# Autodesk Inventor assembly: Servo-Arm-20mm-Ball-Joint
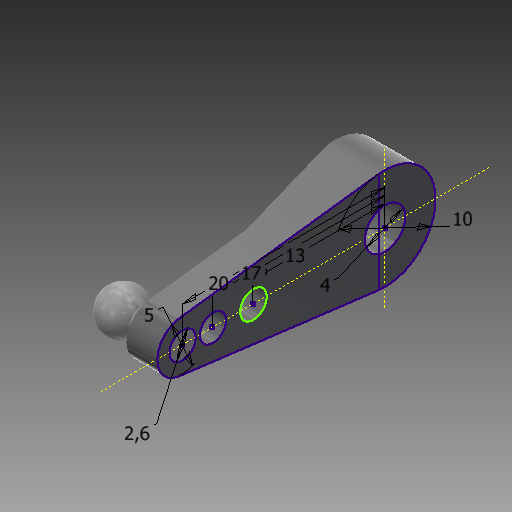
[picture p0: Inventor's stored thumbnail of the model, 512x512]
Saved by Autodesk Inventor 2018.2 (Build 222227000, 227)
## iProperties
Created: 2018-02-23
Part Number: Servo-Arm-20mm-Ball-Joint
Material: Generisch
Document SubType Name: Assembly
Designer: JochenAlt
Author: JochenAlt
## Documents named in this file (3)
- D:\Projects\Donna\CAD\Hitec-5065MG\Servo-Arm-20mm-Ball-Joint.iam
- D:\Projects\Donna\CAD\Hitec-5065MG\Servo-Arm-20mm.ipt
- D:\Projects\Donna\CAD\Hitec-5065MG\Ball-Joint-male.ipt
## Components (2 placed, 2 different names)
1. ServoArm:1 — Passend:1, Passend:2, Passend:3, Passend:4, Passend:5
2. ball joint:1 — Passend:1, Passend:2
## Relationships (5: Mate 5)
- Passend:1 [Mate]: ServoArm:1 ↔ ball joint:1
- Passend:2 [Mate]: ServoArm:1 ↔ ball joint:1
- Passend:3 [Mate]: ServoArm:1
- Passend:4 [Mate]: ServoArm:1
- Passend:5 [Mate]: ServoArm:1
